# Autodesk Inventor assembly: BridgeCar
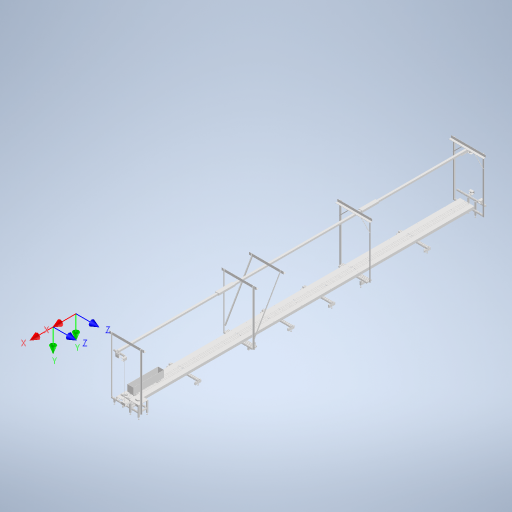
[picture p0: Inventor's stored thumbnail of the model, 512x512]
Saved by Autodesk Inventor 2023 (Build 270158030, 158C)
## iProperties
Created: 2023-02-16
Part Number: BridgeCar
Document SubType Name: Assembly
Designer: jeremyy
Author: jeremyy
## Documents named in this file (3)
- \\andrew.ad.cmu.edu\users\users1\jeremyy\Documents\Inventor\CMU Bridge\New folder\BridgeCar.iam
- \\andrew.ad.cmu.edu\users\users1\jeremyy\Documents\Inventor\CMU Bridge\New folder\Full Bridge.iam
- \\andrew.ad.cmu.edu\users\users1\jeremyy\Documents\Inventor\CMU Bridge\Car\Full Car.iam
## Components (2 placed, 2 different names)
1. Full Bridge:1 [sub-assembly] — Tangent:1, Mate:1, Mate:2
2. Full Car:1 [sub-assembly] — Tangent:1, Mate:1, Mate:2
## Relationships (3: Mate 2, Tangent 1)
- Tangent:1: Full Bridge:1 ↔ Full Car:1
- Mate:1: Full Bridge:1 ↔ Full Car:1
- Mate:2 (127 mm): Full Bridge:1 ↔ Full Car:1
